# Autodesk Inventor assembly: Weapon Assembly
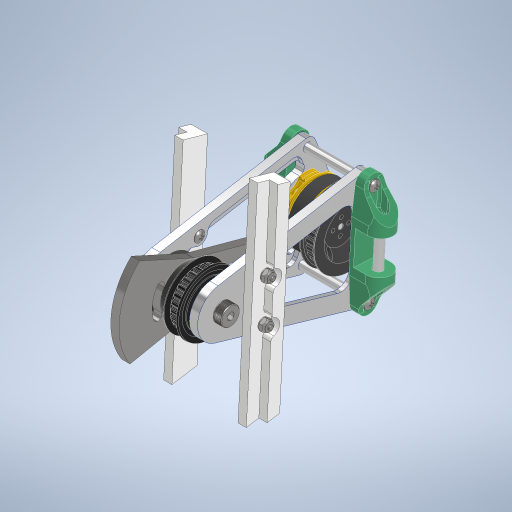
[picture p0: Inventor's stored thumbnail of the model, 512x512]
Saved by Autodesk Inventor 2023.2 (Build 272271000, 271)
## iProperties
Created: 2022-05-21
Part Number: Weapon Assembly
Document SubType Name: Assembly
Designer: Nathan Cai
Mass: 622.735 g
Surface Area: 1390.16 cm^2
Volume: 228.863 cm^3
Density: 2.72099 g/cm^3
Author: Nathan Cai
## Documents named in this file (15)
- C:\Users\Nathan Cai\Documents\Inventor\0.3rd Lawette - V3.6\Vertical Weapon Assembly (Type A - Low Power)\Weapon Assembly (Vert A - Low Power).iam
- C:\Users\Nathan Cai\Documents\Inventor\0.3rd Lawette - V3.6\Vertical Weapon Assembly (Type A)\90807A139_Same-Size Thread Alloy Steel Shoulder Screw.ipt
- C:\Users\Nathan Cai\Documents\Inventor\0.3rd Lawette - V3.6\Vertical Weapon Assembly (Type A)\90630A121_High-Strength Steel Nylon-Insert Locknut.ipt
- C:\Users\Nathan Cai\Documents\Inventor\0.3rd Lawette - V3.6\Standoff 1.5in.ipt
- C:\Users\Nathan Cai\Documents\Inventor\0.3rd Lawette - V3.6\Vertical Weapon Assembly (Type A)\Legs.ipt
- C:\Users\Nathan Cai\Documents\Inventor\Content Center Files\R2023\en-US\ANSI B18.6.3(27)\ANSI B18.6.3 - 6-32 UNC - 0.75(11).ipt
- C:\Users\Nathan Cai\Documents\Inventor\Content Center Files\R2023\en-US\SAE J773b\SAE J773b - No. 6. SAE Type L. narrow.ipt
- C:\Users\Nathan Cai\Documents\Inventor\Content Center Files\R2023\en-US\IFI 100 107(2)\IFI 100_107 - No. 6 - 32 Metal Type.ipt
- C:\Users\Nathan Cai\Documents\Inventor\0.3rd Lawette - V3.6\Vertical Weapon Assembly (Type A)\Legs_MIR.ipt
- C:\Users\Nathan Cai\Documents\Inventor\Content Center Files\R2023\en-US\ANSI B18.6.3(27)\ANSI B18.6.3 - 6-32 UNC - 0.625(11).ipt
- C:\Users\Nathan Cai\Documents\Inventor\0.3rd Lawette - V3.6\Vertical Weapon Assembly (Type A - Low Power)\Weapon (Weapon-Side Pulley).iam
- C:\Users\Nathan Cai\Documents\Inventor\0.3rd Lawette - V3.6\Vertical Weapon Assembly (Type A - Low Power)\Weapon (Motor-Side Pulley).iam
- C:\Users\Nathan Cai\Documents\Inventor\0.3rd Lawette - V3.6\Vertical Weapon Assembly (Type A - Low Power)\Frame (Clear Side).ipt
- C:\Users\Nathan Cai\Documents\Inventor\0.3rd Lawette - V3.6\Vertical Weapon Assembly (Type A - Low Power)\Frame (Motor Side).ipt
- C:\Users\Nathan Cai\Documents\Inventor\0.3rd Lawette - V3.6\Vertical Weapon Assembly (Type A - Low Power)\Bracket.ipt
## Components (42 placed, 14 different names)
1. Weapon (Weapon-Side Pulley):2 [sub-assembly] — Mate:103
2. Weapon (Motor-Side Pulley):2 [sub-assembly] — Mate:167, Mate:226
3. 90807A139_Same-Size Thread Alloy Steel Shoulder Screw:1 — Mate:1, Mate:2
4. 90630A121_High-Strength Steel Nylon-Insert Locknut:1 — Mate:1, Mate:2
5. Frame (Motor Side):2 — Mate:103, Mate:167, Mate:226
6. Frame (Clear Side):2
7. Legs:1 — Mate:207, Mate:209
8. Legs_MIR:1 — Mate:199, Mate:201
9. Bracket:3
10. Bracket:4
11. Standoff 1.5in:1
12. Standoff 1.5in:2
13. Standoff 1.5in:3 — Mate:223, Mate:225
14. Standoff 1.5in:4
15. Cross Recessed Truss Head Machine Screw - Type I - Inch No. 6 - 32 - 5/8:8 — Insert:44
16. Conical Spring Washer SAE J773b (Inch) No. 6. SAE Type L. narrow:38 — Mate:225, Insert:44
17. Cross Recessed Truss Head Machine Screw - Type I - Inch No. 6 - 32 - 5/8:7 — Insert:43
18. Conical Spring Washer SAE J773b (Inch) No. 6. SAE Type L. narrow:37 — Mate:223, Insert:43
19. Cross Recessed Truss Head Machine Screw - Type I - Inch No. 6 - 32 - 5/8:6 — Insert:42
20. Conical Spring Washer SAE J773b (Inch) No. 6. SAE Type L. narrow:36 — Insert:42
21. Cross Recessed Truss Head Machine Screw - Type I - Inch No. 6 - 32 - 5/8:5 — Insert:41
22. Conical Spring Washer SAE J773b (Inch) No. 6. SAE Type L. narrow:35 — Insert:41
23. Cross Recessed Truss Head Machine Screw - Type I - Inch No. 6 - 32 - 3/4:27 — Insert:40
24. Conical Spring Washer SAE J773b (Inch) No. 6. SAE Type L. narrow:34 — Insert:40
25. Cross Recessed Truss Head Machine Screw - Type I - Inch No. 6 - 32 - 3/4:26 — Insert:39
26. Conical Spring Washer SAE J773b (Inch) No. 6. SAE Type L. narrow:33 — Insert:39
27. Cross Recessed Truss Head Machine Screw - Type I - Inch No. 6 - 32 - 3/4:25 — Insert:38
28. Conical Spring Washer SAE J773b (Inch) No. 6. SAE Type L. narrow:32 — Insert:38
29. Cross Recessed Truss Head Machine Screw - Type I - Inch No. 6 - 32 - 3/4:24 — Insert:37
30. Conical Spring Washer SAE J773b (Inch) No. 6. SAE Type L. narrow:31 — Insert:37
31. Prevailing Torque Type Hex Nut - Inch (IFI) No. 6 - 32 Metal Type:22 — Insert:36
32. Conical Spring Washer SAE J773b (Inch) No. 6. SAE Type L. narrow:30 — Mate:209, Insert:36
33. Cross Recessed Truss Head Machine Screw - Type I - Inch No. 6 - 32 - 3/4:23
34. Prevailing Torque Type Hex Nut - Inch (IFI) No. 6 - 32 Metal Type:21 — Insert:35
35. Conical Spring Washer SAE J773b (Inch) No. 6. SAE Type L. narrow:29 — Mate:207, Insert:35
36. Cross Recessed Truss Head Machine Screw - Type I - Inch No. 6 - 32 - 3/4:22
37. Prevailing Torque Type Hex Nut - Inch (IFI) No. 6 - 32 Metal Type:20 — Insert:34
38. Conical Spring Washer SAE J773b (Inch) No. 6. SAE Type L. narrow:28 — Mate:201, Insert:34
39. Cross Recessed Truss Head Machine Screw - Type I - Inch No. 6 - 32 - 3/4:21
40. Prevailing Torque Type Hex Nut - Inch (IFI) No. 6 - 32 Metal Type:19 — Insert:33
41. Conical Spring Washer SAE J773b (Inch) No. 6. SAE Type L. narrow:27 — Mate:199, Insert:33
42. Cross Recessed Truss Head Machine Screw - Type I - Inch No. 6 - 32 - 3/4:20
## Relationships (76: Mate 61, Insert 12, Flush 2, Symmetry 1)
- Mate:1: 90807A139_Same-Size Thread Alloy Steel Shoulder Screw:1 ↔ 90630A121_High-Strength Steel Nylon-Insert Locknut:1
- Mate:2 (50.8 mm): 90807A139_Same-Size Thread Alloy Steel Shoulder Screw:1 ↔ 90630A121_High-Strength Steel Nylon-Insert Locknut:1
- [Mate]: Weapon (Weapon-Side Pulley):2 ↔ 90807A139_Same-Size Thread Alloy Steel Shoulder Screw:1
- [Mate]: 90807A139_Same-Size Thread Alloy Steel Shoulder Screw:1 ↔ Frame (Motor Side):2
- [Mate]: 90807A139_Same-Size Thread Alloy Steel Shoulder Screw:1 ↔ Frame (Clear Side):2
- [Mate]: 90807A139_Same-Size Thread Alloy Steel Shoulder Screw:1 ↔ Frame (Clear Side):2
- [Mate]: Frame (Motor Side):2 ↔ Frame (Clear Side):2
- [Mate]: Frame (Motor Side):2 ↔ Standoff 1.5in:1
- [Mate]: Frame (Motor Side):2 ↔ Standoff 1.5in:2
- [Mate]: Frame (Motor Side):2 ↔ Standoff 1.5in:1
- [Mate]: Frame (Motor Side):2 ↔ Standoff 1.5in:2
- [Mate]: Frame (Clear Side):2 ↔ Legs:1
- [Mate]: Frame (Clear Side):2 ↔ Legs:1
- [Mate]: Frame (Clear Side):2 ↔ Legs:1
- [Mate]: Frame (Clear Side):2 ↔ Standoff 1.5in:1
- Mate:103 (0.0254 mm): Weapon (Weapon-Side Pulley):2 ↔ Frame (Motor Side):2
- [Symmetry]: Frame (Motor Side):2 ↔ Frame (Clear Side):2
- [Mate]: Frame (Motor Side):2 ↔ Legs_MIR:1
- [Mate]: Frame (Motor Side):2 ↔ Legs_MIR:1
- [Mate]: Frame (Motor Side):2 ↔ Legs_MIR:1
- Mate:167: Weapon (Motor-Side Pulley):2 ↔ Frame (Motor Side):2
- [Mate]: Frame (Motor Side):2 ↔ Bracket:4
- [Mate]: Bracket:4 ↔ Standoff 1.5in:1
- [Mate]: Bracket:4 ↔ Standoff 1.5in:2
- [Mate]: Frame (Clear Side):2 ↔ Bracket:3
- [Mate]: Bracket:3 ↔ Standoff 1.5in:1
- [Mate]: Bracket:3 ↔ Standoff 1.5in:2
- [Mate]: Bracket:3 ↔ Standoff 1.5in:3
- [Mate]: Bracket:4 ↔ Standoff 1.5in:4
- [Flush]: Bracket:4 ↔ Standoff 1.5in:4
- [Flush]: Bracket:3 ↔ Standoff 1.5in:3
- [Mate]: Frame (Motor Side):2 ↔ Cross Recessed Truss Head Machine Screw - Type I - Inch No. 6 - 32 - 3/4:20
- [Mate]: Frame (Motor Side):2 ↔ Cross Recessed Truss Head Machine Screw - Type I - Inch No. 6 - 32 - 3/4:20
- [Mate]: Frame (Motor Side):2 ↔ Cross Recessed Truss Head Machine Screw - Type I - Inch No. 6 - 32 - 3/4:21
- [Mate]: Frame (Motor Side):2 ↔ Cross Recessed Truss Head Machine Screw - Type I - Inch No. 6 - 32 - 3/4:21
- [Mate]: Frame (Motor Side):2 ↔ Conical Spring Washer SAE J773b (Inch) No. 6. SAE Type L. narrow:27
- Mate:199: Legs_MIR:1 ↔ Conical Spring Washer SAE J773b (Inch) No. 6. SAE Type L. narrow:27
- [Mate]: Frame (Motor Side):2 ↔ Conical Spring Washer SAE J773b (Inch) No. 6. SAE Type L. narrow:28
- Mate:201: Legs_MIR:1 ↔ Conical Spring Washer SAE J773b (Inch) No. 6. SAE Type L. narrow:28
- Insert:33: Prevailing Torque Type Hex Nut - Inch (IFI) No. 6 - 32 Metal Type:19 ↔ Conical Spring Washer SAE J773b (Inch) No. 6. SAE Type L. narrow:27
- Insert:34: Prevailing Torque Type Hex Nut - Inch (IFI) No. 6 - 32 Metal Type:20 ↔ Conical Spring Washer SAE J773b (Inch) No. 6. SAE Type L. narrow:28
- [Mate]: Frame (Clear Side):2 ↔ Cross Recessed Truss Head Machine Screw - Type I - Inch No. 6 - 32 - 3/4:22
- [Mate]: Frame (Clear Side):2 ↔ Cross Recessed Truss Head Machine Screw - Type I - Inch No. 6 - 32 - 3/4:22
- [Mate]: Frame (Clear Side):2 ↔ Cross Recessed Truss Head Machine Screw - Type I - Inch No. 6 - 32 - 3/4:23
- [Mate]: Frame (Clear Side):2 ↔ Cross Recessed Truss Head Machine Screw - Type I - Inch No. 6 - 32 - 3/4:23
- [Mate]: Frame (Clear Side):2 ↔ Conical Spring Washer SAE J773b (Inch) No. 6. SAE Type L. narrow:29
- Mate:207: Legs:1 ↔ Conical Spring Washer SAE J773b (Inch) No. 6. SAE Type L. narrow:29
- [Mate]: Frame (Clear Side):2 ↔ Conical Spring Washer SAE J773b (Inch) No. 6. SAE Type L. narrow:30
- Mate:209: Legs:1 ↔ Conical Spring Washer SAE J773b (Inch) No. 6. SAE Type L. narrow:30
- Insert:35: Prevailing Torque Type Hex Nut - Inch (IFI) No. 6 - 32 Metal Type:21 ↔ Conical Spring Washer SAE J773b (Inch) No. 6. SAE Type L. narrow:29
- Insert:36: Prevailing Torque Type Hex Nut - Inch (IFI) No. 6 - 32 Metal Type:22 ↔ Conical Spring Washer SAE J773b (Inch) No. 6. SAE Type L. narrow:30
- [Mate]: Bracket:3 ↔ Conical Spring Washer SAE J773b (Inch) No. 6. SAE Type L. narrow:31
- [Mate]: Bracket:3 ↔ Conical Spring Washer SAE J773b (Inch) No. 6. SAE Type L. narrow:31
- [Mate]: Bracket:3 ↔ Conical Spring Washer SAE J773b (Inch) No. 6. SAE Type L. narrow:32
- [Mate]: Bracket:3 ↔ Conical Spring Washer SAE J773b (Inch) No. 6. SAE Type L. narrow:32
- Insert:37: Cross Recessed Truss Head Machine Screw - Type I - Inch No. 6 - 32 - 3/4:24 ↔ Conical Spring Washer SAE J773b (Inch) No. 6. SAE Type L. narrow:31
- Insert:38: Cross Recessed Truss Head Machine Screw - Type I - Inch No. 6 - 32 - 3/4:25 ↔ Conical Spring Washer SAE J773b (Inch) No. 6. SAE Type L. narrow:32
- [Mate]: Bracket:4 ↔ Conical Spring Washer SAE J773b (Inch) No. 6. SAE Type L. narrow:33
- [Mate]: Bracket:4 ↔ Conical Spring Washer SAE J773b (Inch) No. 6. SAE Type L. narrow:33
- [Mate]: Bracket:4 ↔ Conical Spring Washer SAE J773b (Inch) No. 6. SAE Type L. narrow:34
- [Mate]: Bracket:4 ↔ Conical Spring Washer SAE J773b (Inch) No. 6. SAE Type L. narrow:34
- Insert:39: Cross Recessed Truss Head Machine Screw - Type I - Inch No. 6 - 32 - 3/4:26 ↔ Conical Spring Washer SAE J773b (Inch) No. 6. SAE Type L. narrow:33
- Insert:40: Cross Recessed Truss Head Machine Screw - Type I - Inch No. 6 - 32 - 3/4:27 ↔ Conical Spring Washer SAE J773b (Inch) No. 6. SAE Type L. narrow:34
- [Mate]: Bracket:3 ↔ Conical Spring Washer SAE J773b (Inch) No. 6. SAE Type L. narrow:35
- [Mate]: Bracket:3 ↔ Conical Spring Washer SAE J773b (Inch) No. 6. SAE Type L. narrow:35
- [Mate]: Bracket:4 ↔ Conical Spring Washer SAE J773b (Inch) No. 6. SAE Type L. narrow:36
- [Mate]: Bracket:3 ↔ Conical Spring Washer SAE J773b (Inch) No. 6. SAE Type L. narrow:36
- Insert:41: Cross Recessed Truss Head Machine Screw - Type I - Inch No. 6 - 32 - 5/8:5 ↔ Conical Spring Washer SAE J773b (Inch) No. 6. SAE Type L. narrow:35
- Insert:42: Cross Recessed Truss Head Machine Screw - Type I - Inch No. 6 - 32 - 5/8:6 ↔ Conical Spring Washer SAE J773b (Inch) No. 6. SAE Type L. narrow:36
- [Mate]: Bracket:3 ↔ Conical Spring Washer SAE J773b (Inch) No. 6. SAE Type L. narrow:37
- Mate:223: Standoff 1.5in:3 ↔ Conical Spring Washer SAE J773b (Inch) No. 6. SAE Type L. narrow:37
- [Mate]: Bracket:4 ↔ Conical Spring Washer SAE J773b (Inch) No. 6. SAE Type L. narrow:38
- Mate:225: Standoff 1.5in:3 ↔ Conical Spring Washer SAE J773b (Inch) No. 6. SAE Type L. narrow:38
- Insert:43: Cross Recessed Truss Head Machine Screw - Type I - Inch No. 6 - 32 - 5/8:7 ↔ Conical Spring Washer SAE J773b (Inch) No. 6. SAE Type L. narrow:37
- Insert:44: Cross Recessed Truss Head Machine Screw - Type I - Inch No. 6 - 32 - 5/8:8 ↔ Conical Spring Washer SAE J773b (Inch) No. 6. SAE Type L. narrow:38
- Mate:226: Weapon (Motor-Side Pulley):2 ↔ Frame (Motor Side):2
